# Autodesk Inventor assembly: r40
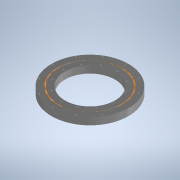
[picture p0: Inventor's stored thumbnail of the model, 180x180]
Saved by Autodesk Inventor 2022 (Build 260153000, 153)
## iProperties
Created: 2022-02-21
Part Number: r40
Document SubType Name: Assembly
Designer: JK
Title: C:/Users/JK/Desktop/r40.step
Sending System: Autodesk Translation Framework v10.13.0.1454
Preprocessor: ST-DEVELOPER v18.1
## Documents named in this file (5)
- C:\Users\JK\Documents\Inventor\ScaraNema\Inverse timing belt reducer\r40.iam
- C:\Users\JK\Documents\Inventor\ScaraNema\Inverse timing belt reducer\Rolls A.ipt
- C:\Users\JK\Documents\Inventor\ScaraNema\Inverse timing belt reducer\Rolls B.ipt
- C:\Users\JK\Documents\Inventor\ScaraNema\Inverse timing belt reducer\Race Outer.ipt
- C:\Users\JK\Documents\Inventor\ScaraNema\Inverse timing belt reducer\Race Inner.ipt
## Components (5 placed, 4 different names)
1. Rolls A:1
2. Rolls B:1
3. Race Outer:1 — Coincidencia:2, Nivelación:1
4. Race Inner:1 — Coincidencia:1, Coincidencia:3, Nivelación:1, Coincidencia:4
5. Race Inner:2 — Coincidencia:1, Coincidencia:2, Coincidencia:3, Coincidencia:4
## Relationships (5: Mate 4, Flush 1)
- Coincidencia:1 [Mate]: Race Inner:1 ↔ Race Inner:2
- Coincidencia:2 [Mate]: Race Outer:1 ↔ Race Inner:2
- Coincidencia:3 [Mate]: Race Inner:1 ↔ Race Inner:2
- Nivelación:1 [Flush]: Race Outer:1 ↔ Race Inner:1
- Coincidencia:4 [Mate]: Race Inner:1 ↔ Race Inner:2
